# Autodesk Inventor assembly: adjustable_double_connector
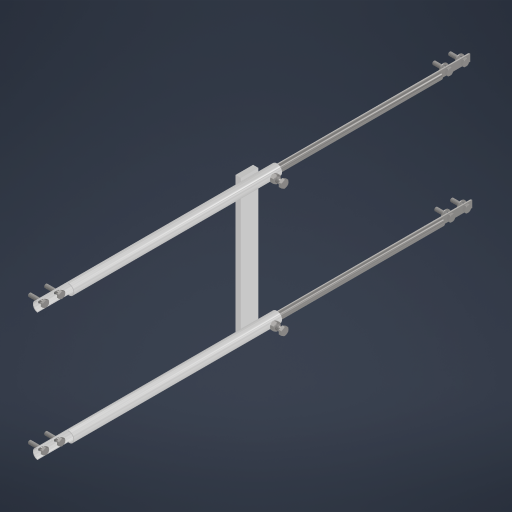
[picture p0: Inventor's stored thumbnail of the model, 512x512]
Saved by Autodesk Inventor 2023 (Build 270158000, 158)
## iProperties
Created: 2022-04-27
Part Number: adjustable_double_connector
Document SubType Name: Assembly
Designer: Norbert Ligas
flat_bar_distance: 15,000 mm
pipe_length: 200,000 mm
iron_angle_to_pipe_edge: 20,000 mm
flat_bar_length: 157,000 mm
flat_bar_thickness: 6,000 mm
flat_bar_width: 20,000 mm
arm_min_length: 11,811 in
arm_max_length: 22,244 in
pipe_inner_diameter: 10,000 mm
pipe_thickness: 1,000 mm
pipe_outer_diameter: 12,000 mm
Author: Norbert Ligas
## Documents named in this file (5)
- C:\Users\norbe\Repozytoria\NormalMapScanner\stand_construction\parts\adjustable_double_connector.iam
- C:\Users\norbe\Repozytoria\NormalMapScanner\stand_construction\parts\adjustable_connector.iam
- C:\Users\norbe\Repozytoria\NormalMapScanner\stand_construction\parts\flat_bar.ipt
- C:\Users\norbe\Repozytoria\NormalMapScanner\stand_construction\parts\adjustable_arm.iam
- C:\Users\norbe\Repozytoria\NormalMapScanner\stand_construction\parts\pipe_connector.ipt
## Components (3 placed, 2 different names)
1. adjustable_connector:1 [sub-assembly] — Flush:1, Angle:1, Tangent:1, Tangent:2, Angle:3
2. adjustable_connector:2 [sub-assembly] — Angle:2, Tangent:3, Tangent:4, Flush:3
3. flat_bar:2 — Flush:1, Flush:2, Tangent:2, Mate:1, Tangent:4, Flush:3, Mate:3, Mate:4, Mate:5, Flush:4
## Relationships (15: Flush 4, Tangent 4, Mate 4, Angle 3)
- Flush:1 (15 mm): adjustable_connector:1 ↔ flat_bar:2
- Angle:1 (0 deg): adjustable_connector:1
- Tangent:1: adjustable_connector:1
- Flush:2: flat_bar:2
- Tangent:2: adjustable_connector:1 ↔ flat_bar:2
- Angle:2 (0 deg): adjustable_connector:2
- Tangent:3: adjustable_connector:2
- Mate:1: flat_bar:2
- Tangent:4: adjustable_connector:2 ↔ flat_bar:2
- Flush:3 (15 mm): adjustable_connector:2 ↔ flat_bar:2
- Mate:3: flat_bar:2
- Mate:4: flat_bar:2
- Mate:5: flat_bar:2
- Angle:3 (0 deg): adjustable_connector:1
- Flush:4: flat_bar:2
## Named parameters: pipe_length = 200 mm, iron_angle_to_pipe_edge = 20 mm, flat_bar_length = 157 mm, flat_bar_thickness = 6 mm, flat_bar_width = 20 mm, flat_bar_distance = 15 mm, arm_min_length = 300 mm, arm_max_length = 565 mm, pipe_inner_diameter = 10 mm, pipe_thickness = 1 mm, pipe_outer_diameter = 12 mm
